# Autodesk Inventor assembly: FY 30 TR
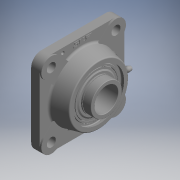
[picture p0: Inventor's stored thumbnail of the model, 180x180]
Saved by Autodesk Inventor 2017.3 (Build 213256000, 256)
## iProperties
Category: PARTsolutions
Company: SKF
Part Number: FY 30 TR
Catalog Web Link: www.cadenas.de
Description: AYF_001HC_HH_HY-Y-bearing square flanged units
Vendor: SKF
Document SubType Name: Assembly
Designer: partserver
Manufacturer: SKF
Mass: 1000 g
Surface Area: 694.379 cm^2
Volume: 145.837 cm^3
Density: 6.85699 g/cm^3
Title: FY 30 TR
Author: Cadenas PARTsolutions
Comments: Y-bearing square flanged units
PSOL_IDENT_0: {$CADENAS_DATA\23d-libs\skf\bearings_units_and_housings\bearing_units\ball_bearing_units\y-units\ayf
PSOL_IDENT_1: _001hc_hh_hy.prj},187 {VTYP=3D},{STYP=ASSTAB},{NB=FY 30 TR},{LINA=FY 30 TR},{NN=AYF_001HC_HH_HY},{DA
PSOL_IDENT_2: TE=20.08.2020 12:22:38},{GEOMDATE=20.08.2020 12:22:32},{VERSION=},{LINEID=52400},{WBVAR=COVER},{WBNU
PSOL_IDENT_3: MERIC=}  {NB=FY 30 TR},{LINA=FY 30 TR},{KT=DUMMY},{DESIGNATION=FY 30 TR},{HOUSING=FY 506 M},{BEARING=
PSOL_IDENT_4: YAR 206-2RF},{COVER=},{DD=30},{DDX=},{DDALG=30.000},{DD1=39.700},{DD2=MIN},{DD3=},{AALG=32.500},{A=3
PSOL_IDENT_5: 2.5},{AX=},{AXX=},{A1ALG=13.000},{A1=13},{A1X=},{A1XX=},{A3ALG=3.200},{A3=3.2},{A3X=},{A5ALG=22.500}
PSOL_IDENT_6: ,{A5=22.5},{A5X=},{A5XX=},{B=38.100},{B1=MIN},{B1X=},{B4ALG=5.000},{B4=5},{B4X=},{DAAALG=93.700},{DA
PSOL_IDENT_7: A=93.7},{DAAX=},{DB=MIN},{DB1=76.000},{DB1X=},{DB2=84.000},{DB2X=},{HA=},{J=82.500},{JX=},{JXX=},{L=
PSOL_IDENT_8: 108.000},{LX=},{LXX=},{N=11.500},{NX=},{NXX=},{SS1=22.200},{SS1X=},{T=42.200},{TX=},{DN=6.500},{SWN=
PSOL_IDENT_9: 7},{GN=1/4-28 SAE-LT},{RG=1/4-28 UNF},{RGX=},{R1=21},{R1X=},{J6=96},{J7=24.500},{N4=4},{D=62.000},{C=
PSOL_IDENT_10: 18.000},{R12=0.600},{DW=9.525},{B3=MIN},{PITCH=46.000},{LOAD1=19.500},{LOAD2=11.200},{LOAD3=0.475},{
PSOL_IDENT_11: SPEED1=3800},{II=1},{Z=9},{MASS=1.000},{MASSX=},{G2=M6x0.75},{HKSGS=3},{RTTGS=4},{ALPHA=},{GALG=10.0
PSOL_IDENT_12: 00},{G=10},{GX=},{GXX=},{GINALG=0.375},{GIN=0.375000002475},{GINX=},{GINXX=},{EC=},{BS=},{SLEEVE=},{
PSOL_IDENT_13: POPULAR=},{D1=MIN},{K=1.7},{CC1=5.1},{BRGTYP=BBY_006},{COVERALG=  '', 'No end cover' },{SUPPRESSED=u
PSOL_IDENT_14: nsuppressed},{TC=FY 30 TR},{PPATH=y-bearing_square_flanged_units_parts/ayf_001hc_hh_hy_asmtpl.prj}
NB: FY 30 TR
NN: AYF_001HC_HH_HY
NT: Y-bearing square flanged units
NBSYN: $TC.
LINA: FY 30 TR
CATALOG: SKF
DESIGNATION: FY 30 TR
HOUSING: FY 506 M
BEARING: YAR 206-2RF
COVER: No end cover
DDALG: 30
J: 82.5
L: 108
T: 42.2
LOAD1: 19.5
LOAD2: 11.2
SPEED1: 3800
SUPPLIER: SKF
ARTICLENO: FY 30 TR
BOMINFO: FY 30 TR
CREATOR: CADENAS GmbH
## Documents named in this file (6)
- e:\temp\worker_92\temp\exporttempdir_8364_58_eTQXT\format_0\FY 30 TR.iam
- e:\temp\worker_92\temp\exporttempdir_8364_58_eTQXT\format_0\FY 30 TR0_375000002475-dummy.ipt
- e:\temp\worker_92\temp\exporttempdir_8364_58_eTQXT\format_0\FY 506 M-housing.ipt
- e:\temp\worker_92\temp\exporttempdir_8364_58_eTQXT\format_0\1_4-28 SAE-LT.ipt
- e:\temp\worker_92\temp\exporttempdir_8364_58_eTQXT\format_0\YAR 206-2RF-39_710300320618 -bearing.ipt
- e:\temp\worker_92\temp\exporttempdir_8364_58_eTQXT\format_0\30-62-38_1-18-ybrg1-61-9_525-46.ipt
## Components (13 placed, 5 different names)
1. FY 30 TR0_375000002475-dummy:1 — brg_XY@1 <-> housing_XY@2, brg_Z@1 <-> housing_Z@2, brg_YZ@1 <-> housing_YZ@2
2. FY 506 M-housing:1 — brg_XY@1 <-> housing_XY@2, brg_Z@1 <-> housing_Z@2, brg_YZ@1 <-> housing_YZ@2, gn_XY@2 <-> gn_XY@3, gn_Z@2 <-> gn_Z@3, gn_YZ@2 <-> gn_YZ@3, housing_XY@2 <-> brg3_XY@4, housing_Z@2 <-> brg3_Z@4, housing_YZ@2 <-> brg3_YZ@4
3. 1_4-28 SAE-LT:1 — gn_XY@2 <-> gn_XY@3, gn_Z@2 <-> gn_Z@3, gn_YZ@2 <-> gn_YZ@3
4. YAR 206-2RF-39_710300320618 -bearing:1 — housing_XY@2 <-> brg3_XY@4, housing_Z@2 <-> brg3_Z@4, housing_YZ@2 <-> brg3_YZ@4, ball_1_XY@4 <-> ball_XY@5, ball_1_Z@4 <-> ball_Z@5, ball_1_YZ@4 <-> ball_YZ@5, ball_2_XY@4 <-> ball_XY@6, ball_2_Z@4 <-> ball_Z@6, ball_2_YZ@4 <-> ball_YZ@6, ball_3_XY@4 <-> ball_XY@7, ball_3_Z@4 <-> ball_Z@7, ball_3_YZ@4 <-> ball_YZ@7, ball_4_XY@4 <-> ball_XY@8, ball_4_Z@4 <-> ball_Z@8, ball_4_YZ@4 <-> ball_YZ@8, ball_5_XY@4 <-> ball_XY@9, ball_5_Z@4 <-> ball_Z@9, ball_5_YZ@4 <-> ball_YZ@9, ball_6_XY@4 <-> ball_XY@10, ball_6_Z@4 <-> ball_Z@10, ball_6_YZ@4 <-> ball_YZ@10, ball_7_XY@4 <-> ball_XY@11, ball_7_Z@4 <-> ball_Z@11, ball_7_YZ@4 <-> ball_YZ@11, ball_8_XY@4 <-> ball_XY@12, ball_8_Z@4 <-> ball_Z@12, ball_8_YZ@4 <-> ball_YZ@12, ball_9_XY@4 <-> ball_XY@13, ball_9_Z@4 <-> ball_Z@13, ball_9_YZ@4 <-> ball_YZ@13
5. 30-62-38_1-18-ybrg1-61-9_525-46:1 — ball_1_XY@4 <-> ball_XY@5, ball_1_Z@4 <-> ball_Z@5, ball_1_YZ@4 <-> ball_YZ@5
6. 30-62-38_1-18-ybrg1-61-9_525-46:2 — ball_2_XY@4 <-> ball_XY@6, ball_2_Z@4 <-> ball_Z@6, ball_2_YZ@4 <-> ball_YZ@6
7. 30-62-38_1-18-ybrg1-61-9_525-46:3 — ball_3_XY@4 <-> ball_XY@7, ball_3_Z@4 <-> ball_Z@7, ball_3_YZ@4 <-> ball_YZ@7
8. 30-62-38_1-18-ybrg1-61-9_525-46:4 — ball_4_XY@4 <-> ball_XY@8, ball_4_Z@4 <-> ball_Z@8, ball_4_YZ@4 <-> ball_YZ@8
9. 30-62-38_1-18-ybrg1-61-9_525-46:5 — ball_5_XY@4 <-> ball_XY@9, ball_5_Z@4 <-> ball_Z@9, ball_5_YZ@4 <-> ball_YZ@9
10. 30-62-38_1-18-ybrg1-61-9_525-46:6 — ball_6_XY@4 <-> ball_XY@10, ball_6_Z@4 <-> ball_Z@10, ball_6_YZ@4 <-> ball_YZ@10
11. 30-62-38_1-18-ybrg1-61-9_525-46:7 — ball_7_XY@4 <-> ball_XY@11, ball_7_Z@4 <-> ball_Z@11, ball_7_YZ@4 <-> ball_YZ@11
12. 30-62-38_1-18-ybrg1-61-9_525-46:8 — ball_8_XY@4 <-> ball_XY@12, ball_8_Z@4 <-> ball_Z@12, ball_8_YZ@4 <-> ball_YZ@12
13. 30-62-38_1-18-ybrg1-61-9_525-46:9 — ball_9_XY@4 <-> ball_XY@13, ball_9_Z@4 <-> ball_Z@13, ball_9_YZ@4 <-> ball_YZ@13
## Relationships (36: Mate 23, Angle 12, Flush 1)
- brg_XY@1 <-> housing_XY@2 [Mate]: FY 30 TR0_375000002475-dummy:1 ↔ FY 506 M-housing:1
- brg_Z@1 <-> housing_Z@2 [Mate]: FY 30 TR0_375000002475-dummy:1 ↔ FY 506 M-housing:1
- brg_YZ@1 <-> housing_YZ@2 [Angle] (180 deg): FY 30 TR0_375000002475-dummy:1 ↔ FY 506 M-housing:1
- gn_XY@2 <-> gn_XY@3 [Mate]: FY 506 M-housing:1 ↔ 1_4-28 SAE-LT:1
- gn_Z@2 <-> gn_Z@3 [Mate]: FY 506 M-housing:1 ↔ 1_4-28 SAE-LT:1
- gn_YZ@2 <-> gn_YZ@3 [Angle] (0 deg): FY 506 M-housing:1 ↔ 1_4-28 SAE-LT:1
- housing_XY@2 <-> brg3_XY@4 [Flush] (42.2 mm): FY 506 M-housing:1 ↔ YAR 206-2RF-39_710300320618 -bearing:1
- housing_Z@2 <-> brg3_Z@4 [Mate]: FY 506 M-housing:1 ↔ YAR 206-2RF-39_710300320618 -bearing:1
- housing_YZ@2 <-> brg3_YZ@4 [Angle] (0 deg): FY 506 M-housing:1 ↔ YAR 206-2RF-39_710300320618 -bearing:1
- ball_1_XY@4 <-> ball_XY@5 [Mate]: YAR 206-2RF-39_710300320618 -bearing:1 ↔ 30-62-38_1-18-ybrg1-61-9_525-46:1
- ball_1_Z@4 <-> ball_Z@5 [Mate]: YAR 206-2RF-39_710300320618 -bearing:1 ↔ 30-62-38_1-18-ybrg1-61-9_525-46:1
- ball_1_YZ@4 <-> ball_YZ@5 [Angle] (0 deg): YAR 206-2RF-39_710300320618 -bearing:1 ↔ 30-62-38_1-18-ybrg1-61-9_525-46:1
- ball_2_XY@4 <-> ball_XY@6 [Mate]: YAR 206-2RF-39_710300320618 -bearing:1 ↔ 30-62-38_1-18-ybrg1-61-9_525-46:2
- ball_2_Z@4 <-> ball_Z@6 [Mate]: YAR 206-2RF-39_710300320618 -bearing:1 ↔ 30-62-38_1-18-ybrg1-61-9_525-46:2
- ball_2_YZ@4 <-> ball_YZ@6 [Angle] (0 deg): YAR 206-2RF-39_710300320618 -bearing:1 ↔ 30-62-38_1-18-ybrg1-61-9_525-46:2
- ball_3_XY@4 <-> ball_XY@7 [Mate]: YAR 206-2RF-39_710300320618 -bearing:1 ↔ 30-62-38_1-18-ybrg1-61-9_525-46:3
- ball_3_Z@4 <-> ball_Z@7 [Mate]: YAR 206-2RF-39_710300320618 -bearing:1 ↔ 30-62-38_1-18-ybrg1-61-9_525-46:3
- ball_3_YZ@4 <-> ball_YZ@7 [Angle] (0 deg): YAR 206-2RF-39_710300320618 -bearing:1 ↔ 30-62-38_1-18-ybrg1-61-9_525-46:3
- ball_4_XY@4 <-> ball_XY@8 [Mate]: YAR 206-2RF-39_710300320618 -bearing:1 ↔ 30-62-38_1-18-ybrg1-61-9_525-46:4
- ball_4_Z@4 <-> ball_Z@8 [Mate]: YAR 206-2RF-39_710300320618 -bearing:1 ↔ 30-62-38_1-18-ybrg1-61-9_525-46:4
- ball_4_YZ@4 <-> ball_YZ@8 [Angle] (0 deg): YAR 206-2RF-39_710300320618 -bearing:1 ↔ 30-62-38_1-18-ybrg1-61-9_525-46:4
- ball_5_XY@4 <-> ball_XY@9 [Mate]: YAR 206-2RF-39_710300320618 -bearing:1 ↔ 30-62-38_1-18-ybrg1-61-9_525-46:5
- ball_5_Z@4 <-> ball_Z@9 [Mate]: YAR 206-2RF-39_710300320618 -bearing:1 ↔ 30-62-38_1-18-ybrg1-61-9_525-46:5
- ball_5_YZ@4 <-> ball_YZ@9 [Angle] (0 deg): YAR 206-2RF-39_710300320618 -bearing:1 ↔ 30-62-38_1-18-ybrg1-61-9_525-46:5
- ball_6_XY@4 <-> ball_XY@10 [Mate]: YAR 206-2RF-39_710300320618 -bearing:1 ↔ 30-62-38_1-18-ybrg1-61-9_525-46:6
- ball_6_Z@4 <-> ball_Z@10 [Mate]: YAR 206-2RF-39_710300320618 -bearing:1 ↔ 30-62-38_1-18-ybrg1-61-9_525-46:6
- ball_6_YZ@4 <-> ball_YZ@10 [Angle] (0 deg): YAR 206-2RF-39_710300320618 -bearing:1 ↔ 30-62-38_1-18-ybrg1-61-9_525-46:6
- ball_7_XY@4 <-> ball_XY@11 [Mate]: YAR 206-2RF-39_710300320618 -bearing:1 ↔ 30-62-38_1-18-ybrg1-61-9_525-46:7
- ball_7_Z@4 <-> ball_Z@11 [Mate]: YAR 206-2RF-39_710300320618 -bearing:1 ↔ 30-62-38_1-18-ybrg1-61-9_525-46:7
- ball_7_YZ@4 <-> ball_YZ@11 [Angle] (0 deg): YAR 206-2RF-39_710300320618 -bearing:1 ↔ 30-62-38_1-18-ybrg1-61-9_525-46:7
- ball_8_XY@4 <-> ball_XY@12 [Mate]: YAR 206-2RF-39_710300320618 -bearing:1 ↔ 30-62-38_1-18-ybrg1-61-9_525-46:8
- ball_8_Z@4 <-> ball_Z@12 [Mate]: YAR 206-2RF-39_710300320618 -bearing:1 ↔ 30-62-38_1-18-ybrg1-61-9_525-46:8
- ball_8_YZ@4 <-> ball_YZ@12 [Angle] (0 deg): YAR 206-2RF-39_710300320618 -bearing:1 ↔ 30-62-38_1-18-ybrg1-61-9_525-46:8
- ball_9_XY@4 <-> ball_XY@13 [Mate]: YAR 206-2RF-39_710300320618 -bearing:1 ↔ 30-62-38_1-18-ybrg1-61-9_525-46:9
- ball_9_Z@4 <-> ball_Z@13 [Mate]: YAR 206-2RF-39_710300320618 -bearing:1 ↔ 30-62-38_1-18-ybrg1-61-9_525-46:9
- ball_9_YZ@4 <-> ball_YZ@13 [Angle] (0 deg): YAR 206-2RF-39_710300320618 -bearing:1 ↔ 30-62-38_1-18-ybrg1-61-9_525-46:9
